# Autodesk Inventor assembly: wirst
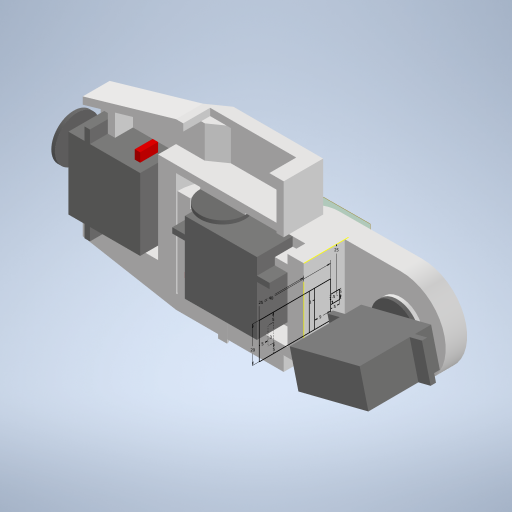
[picture p0: Inventor's stored thumbnail of the model, 512x512]
Saved by Autodesk Inventor 2023 (Build 270158000, 158)
## iProperties
Created: 2024-06-27
Part Number: wirst
Document SubType Name: Assembly
Designer: Swoby
Author: Swoby
## Documents named in this file (5)
- C:\Users\Swoby\OneDrive\Plocha\DUM-E\V0.2\wirst.iam
- C:\Users\Swoby\OneDrive\Plocha\DUM-E\V0.2\Servo_bigg_top.ipt
- C:\Users\Swoby\OneDrive\Plocha\DUM-E\V0.2\Servo_bigg_maketa.ipt
- C:\Users\Swoby\OneDrive\Plocha\DUM-E\V0.2\wirst 1 left.ipt
- C:\Users\Swoby\OneDrive\Plocha\DUM-E\V0.2\wirst 2 right.ipt
## Components (8 placed, 4 different names)
1. Servo_bigg_top:1 — Mate:1, Mate:2
2. Servo_bigg_maketa:1 — Mate:1, Mate:2, Mate:3, Mate:4, Mate:5
3. wirst 1 left:1 — Mate:3, Mate:4, Mate:5, Mate:11, Mate:12
4. wirst 2 right:1 — Mate:6, Mate:7, Mate:8, Mate:15, Mate:16
5. Servo_bigg_top:2 — Mate:9, Mate:10, Mate:11, Mate:12
6. Servo_bigg_maketa:2 — Mate:6, Mate:7, Mate:8, Mate:9, Mate:10
7. Servo_bigg_top:3 — Mate:13, Mate:14, Mate:15, Mate:16
8. Servo_bigg_maketa:3 — Mate:13, Mate:14
## Relationships (16: Mate 16)
- Mate:1: Servo_bigg_top:1 ↔ Servo_bigg_maketa:1
- Mate:2: Servo_bigg_top:1 ↔ Servo_bigg_maketa:1
- Mate:3: Servo_bigg_maketa:1 ↔ wirst 1 left:1
- Mate:4: Servo_bigg_maketa:1 ↔ wirst 1 left:1
- Mate:5: Servo_bigg_maketa:1 ↔ wirst 1 left:1
- Mate:6: wirst 2 right:1 ↔ Servo_bigg_maketa:2
- Mate:7: wirst 2 right:1 ↔ Servo_bigg_maketa:2
- Mate:8: wirst 2 right:1 ↔ Servo_bigg_maketa:2
- Mate:9: Servo_bigg_top:2 ↔ Servo_bigg_maketa:2
- Mate:10: Servo_bigg_top:2 ↔ Servo_bigg_maketa:2
- Mate:11: wirst 1 left:1 ↔ Servo_bigg_top:2
- Mate:12: wirst 1 left:1 ↔ Servo_bigg_top:2
- Mate:13: Servo_bigg_top:3 ↔ Servo_bigg_maketa:3
- Mate:14: Servo_bigg_top:3 ↔ Servo_bigg_maketa:3
- Mate:15: wirst 2 right:1 ↔ Servo_bigg_top:3
- Mate:16: wirst 2 right:1 ↔ Servo_bigg_top:3
